# Autodesk Inventor assembly: MG996R SBORKA
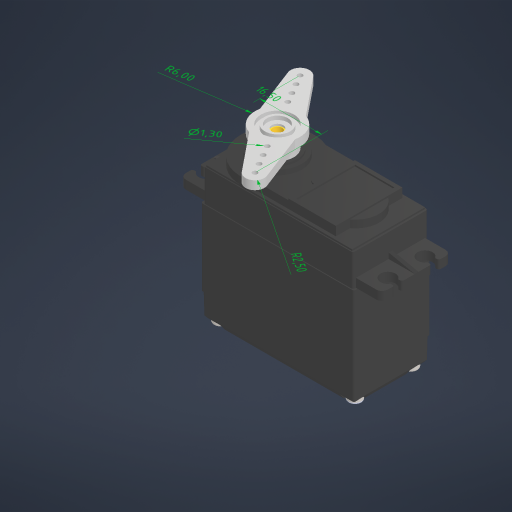
[picture p0: Inventor's stored thumbnail of the model, 512x512]
Saved by Autodesk Inventor 2024 (Build 280153000, 153)
## iProperties
Created: 2020-10-15
Part Number: MG996R SBORKA
Document SubType Name: Assembly
Designer: user
Sending System: SolidWorks 2017
Last Author: Alien
Last Saved: 2021-01-24
Author: user
## Documents named in this file (4)
- D:\Docs\Robot\3d\electronics\servo\MG996R SBORKA.iam
- D:\Docs\Robot\3d\electronics\servo\MG996R SBORKA\Servo MG996R.ipt
- D:\Docs\Robot\3d\electronics\servo\MG996R SBORKA\Servo MG996R Shaft.ipt
- D:\Docs\Robot\3d\electronics\servo\MG996R SBORKA\Servo MG996R arm01.ipt
## Components (3 placed, 3 different names)
1. Servo MG996R:1 — Вставка:1, Вставка:2, Угол:1
2. Servo MG996R Shaft:1 — Вставка:1
3. Servo MG996R arm01:1 — Вставка:2, Угол:1
## Relationships (3: Insert 2, Angle 1)
- Вставка:1 [Insert]: Servo MG996R:1 ↔ Servo MG996R Shaft:1
- Вставка:2 [Insert]: Servo MG996R:1 ↔ Servo MG996R arm01:1
- Угол:1 [Angle] (-30 deg): Servo MG996R:1 ↔ Servo MG996R arm01:1
